# Autodesk Inventor assembly: MultiPass0V_outsideIn-DFMOD
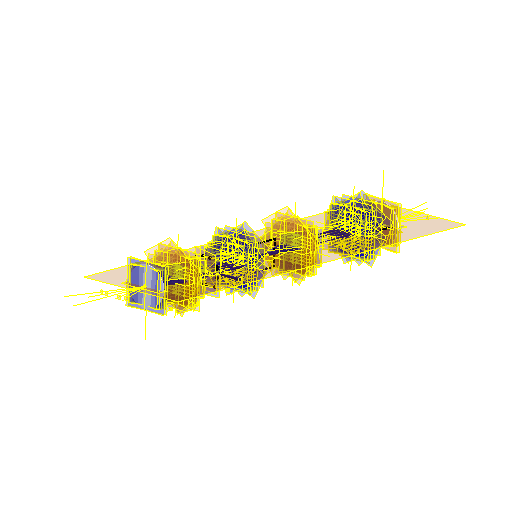
[picture p0: Inventor's stored thumbnail of the model, 512x512]
Saved by Autodesk Inventor 2026.1 (Build 301233000, 233)
## iProperties
Created: 2024-08-19
Part Number: MultiPass0V_outsideIn-DFMOD
Document SubType Name: Assembly
Designer: User
Author: User
## Documents named in this file (14)
- C:\Users\farin012\Downloads\fig4\fig4\MultiPass0V_outsideIn-DFMOD.iam
- C:\Users\farin012\Downloads\fig4\fig4\BB1-E02-Solidworks.ipt
- C:\Users\farin012\Downloads\fig4\fig4\LaserBeamEntry2.ipt
- C:\Users\farin012\Downloads\fig4\fig4\LoopPlane1.ipt
- C:\Users\farin012\Downloads\fig4\fig4\LA1608-AB-Solidworks\LA1608-AB-2LOOP_grid.ipt
- C:\Users\farin012\Downloads\fig4\fig4\LOOP1_COLL.ipt
- C:\Users\farin012\Downloads\fig4\fig4\LOOP1_COLL_L.ipt
- C:\Users\farin012\Downloads\fig4\fig4\LOOP2_COLL.ipt
- C:\Users\farin012\Downloads\fig4\fig4\LOOP2_COLL_L.ipt
- C:\Users\farin012\Downloads\fig4\fig4\LOOP3_COLL.ipt
- C:\Users\farin012\Downloads\fig4\fig4\LOOP3_COLL_L.ipt
- C:\Users\farin012\Downloads\fig4\fig4\deflection_plane.ipt
- C:\Users\farin012\Downloads\fig4\fig4\ExitMirror.ipt
- C:\Users\farin012\Downloads\fig4\fig4\EntryMirror.ipt
## Components (42 placed, 13 different names)
1. BB1-E02-Solidworks:1 — Mate:115, Mate:125, Mate:126, Mate:127, Angle:6, Mate:128, Mate:147, Mate:157, Mate:158, Mate:159, Mate:160
2. BB1-E02-Solidworks:2 — Angle:5, Mate:137, Mate:138, Mate:191
3. LaserBeamEntry2:16 — Mate:124, Flush:7, Mate:179, Mate:180
4. LoopPlane1:1 — Mate:113
5. LA1608-AB-2LOOP_grid:1 — Flush:3, Mate:124, Flush:7, Flush:8, Mate:129, Mate:145, Mate:147, Mate:148, Mate:156, Flush:15, Mate:161, Flush:16
6. LA1608-AB-2LOOP_grid:2 — Flush:2, Flush:9, Mate:130, Mate:136, Mate:145, Mate:146, Mate:149, Mate:155, Flush:14, Mate:162, Flush:17, Mate:164, Mate:174, Flush:22
7. LA1608-AB-2LOOP_grid:3 — Flush:5, Mate:134, Flush:11, Mate:137, Mate:139, Mate:140, Mate:141, Mate:142, Mate:143, Flush:12, Mate:151, Mate:152, Mate:166, Flush:19, Mate:167, Mate:168, Mate:170, Flush:20
8. LA1608-AB-2LOOP_grid:4 — Flush:4, Mate:133, Flush:10, Mate:135, Mate:144, Flush:13, Mate:146, Mate:150, Mate:152, Mate:153, Mate:154, Mate:163, Mate:165, Flush:18, Flush:21
9. LOOP1_COLL:1 — Mate:125, Mate:126
10. LOOP1_COLL:2 — Mate:127, Mate:128
11. LaserBeamEntry2:17 — Flush:8, Mate:129
12. LaserBeamEntry2:18 — Flush:9, Mate:130
13. LOOP1_COLL_L:1 — Mate:135, Mate:136
14. LaserBeamEntry2:19 — Mate:133, Flush:10
15. LaserBeamEntry2:20 — Mate:134, Flush:11
16. LOOP1_COLL:3 — Mate:139, Mate:140
17. LOOP2_COLL:1 — Mate:141, Mate:142
18. LaserBeamEntry2:21 — Mate:144, Flush:13
19. LaserBeamEntry2:22 — Mate:143, Flush:12
20. LOOP2_COLL_L:1 — Mate:153, Mate:154
21. LaserBeamEntry2:23 — Mate:156, Flush:15
22. LaserBeamEntry2:24 — Mate:155, Flush:14
23. LOOP2_COLL:2 — Mate:157, Mate:158
24. LOOP2_COLL:3 — Mate:159, Mate:160
25. LaserBeamEntry2:25 — Mate:161, Flush:16
26. LaserBeamEntry2:26 — Mate:162, Flush:17
27. LOOP2_COLL_L:2 — Mate:163, Mate:164
28. LaserBeamEntry2:27 — Mate:165, Flush:18
29. LaserBeamEntry2:28 — Mate:166, Flush:19
30. LOOP2_COLL:4 — Mate:167, Mate:168
31. LOOP3_COLL:1 — Mate:169, Mate:170
32. LaserBeamEntry2:29 — Mate:172, Flush:21, Mate:188
33. LaserBeamEntry2:30 — Mate:171, Flush:20
34. LOOP3_COLL_L:1 — Mate:173, Mate:174
35. LaserBeamEntry2:31 — Mate:175, Flush:22
36. deflection_plane:1 — Mate:178, Mate:179, Mate:181, Flush:24
37. deflection_plane:2 — Mate:188, Flush:26, Mate:189
38. ExitMirror:1 — Mate:183, Mate:184, Flush:24, Mate:185, Flush:25, Mate:189
39. EntryMirror:1 — Mate:180, Angle:7, Mate:181, Mate:182, Flush:23
40. LaserBeamEntry2:32 — Mate:182, Flush:23
41. LaserBeamEntry2:33 — Mate:185, Flush:25
42. deflection_plane:3 — Mate:190, Angle:8, Mate:191
## Relationships (94: Mate 66, Flush 24, Angle 4)
- Mate:22
- Mate:23
- Mate:113: LoopPlane1:1
- Mate:115: BB1-E02-Solidworks:1
- Angle:5 (180 deg): BB1-E02-Solidworks:2
- Flush:2: LA1608-AB-2LOOP_grid:2
- Flush:3: LA1608-AB-2LOOP_grid:1
- Flush:4: LA1608-AB-2LOOP_grid:4
- Flush:5: LA1608-AB-2LOOP_grid:3
- Mate:124: LaserBeamEntry2:16 ↔ LA1608-AB-2LOOP_grid:1
- Flush:7: LaserBeamEntry2:16 ↔ LA1608-AB-2LOOP_grid:1
- Mate:125: BB1-E02-Solidworks:1 ↔ LOOP1_COLL:1
- Mate:126: BB1-E02-Solidworks:1 ↔ LOOP1_COLL:1
- Mate:127: BB1-E02-Solidworks:1 ↔ LOOP1_COLL:2
- Angle:6 (0 deg): BB1-E02-Solidworks:1
- Mate:128: BB1-E02-Solidworks:1 ↔ LOOP1_COLL:2
- Flush:8: LA1608-AB-2LOOP_grid:1 ↔ LaserBeamEntry2:17
- Mate:129: LA1608-AB-2LOOP_grid:1 ↔ LaserBeamEntry2:17
- Flush:9: LA1608-AB-2LOOP_grid:2 ↔ LaserBeamEntry2:18
- Mate:130: LA1608-AB-2LOOP_grid:2 ↔ LaserBeamEntry2:18
- Mate:133: LA1608-AB-2LOOP_grid:4 ↔ LaserBeamEntry2:19
- Flush:10: LA1608-AB-2LOOP_grid:4 ↔ LaserBeamEntry2:19
- Mate:134: LA1608-AB-2LOOP_grid:3 ↔ LaserBeamEntry2:20
- Flush:11: LA1608-AB-2LOOP_grid:3 ↔ LaserBeamEntry2:20
- Mate:135: LA1608-AB-2LOOP_grid:4 ↔ LOOP1_COLL_L:1
- Mate:136: LA1608-AB-2LOOP_grid:2 ↔ LOOP1_COLL_L:1
- Mate:137 (25 mm): BB1-E02-Solidworks:2 ↔ LA1608-AB-2LOOP_grid:3
- Mate:138: BB1-E02-Solidworks:2
- Mate:139: LA1608-AB-2LOOP_grid:3 ↔ LOOP1_COLL:3
- Mate:140: LA1608-AB-2LOOP_grid:3 ↔ LOOP1_COLL:3
- Mate:141: LA1608-AB-2LOOP_grid:3 ↔ LOOP2_COLL:1
- Mate:142: LA1608-AB-2LOOP_grid:3 ↔ LOOP2_COLL:1
- Mate:143: LA1608-AB-2LOOP_grid:3 ↔ LaserBeamEntry2:22
- Flush:12: LA1608-AB-2LOOP_grid:3 ↔ LaserBeamEntry2:22
- Mate:144: LA1608-AB-2LOOP_grid:4 ↔ LaserBeamEntry2:21
- Flush:13: LA1608-AB-2LOOP_grid:4 ↔ LaserBeamEntry2:21
- Mate:145 (-50 mm): LA1608-AB-2LOOP_grid:1 ↔ LA1608-AB-2LOOP_grid:2
- Mate:146 (50 mm): LA1608-AB-2LOOP_grid:2 ↔ LA1608-AB-2LOOP_grid:4
- Mate:147 (25 mm): BB1-E02-Solidworks:1 ↔ LA1608-AB-2LOOP_grid:1
- Mate:148: LA1608-AB-2LOOP_grid:1
- Mate:149: LA1608-AB-2LOOP_grid:2
- Mate:150: LA1608-AB-2LOOP_grid:4
- Mate:151: LA1608-AB-2LOOP_grid:3
- Mate:152 (-50 mm): LA1608-AB-2LOOP_grid:3 ↔ LA1608-AB-2LOOP_grid:4
- Mate:153: LA1608-AB-2LOOP_grid:4 ↔ LOOP2_COLL_L:1
- Mate:154: LA1608-AB-2LOOP_grid:4 ↔ LOOP2_COLL_L:1
- Mate:155: LA1608-AB-2LOOP_grid:2 ↔ LaserBeamEntry2:24
- Flush:14: LA1608-AB-2LOOP_grid:2 ↔ LaserBeamEntry2:24
- Mate:156: LA1608-AB-2LOOP_grid:1 ↔ LaserBeamEntry2:23
- Flush:15: LA1608-AB-2LOOP_grid:1 ↔ LaserBeamEntry2:23
- Mate:157: BB1-E02-Solidworks:1 ↔ LOOP2_COLL:2
- Mate:158: BB1-E02-Solidworks:1 ↔ LOOP2_COLL:2
- Mate:159: BB1-E02-Solidworks:1 ↔ LOOP2_COLL:3
- Mate:160: BB1-E02-Solidworks:1 ↔ LOOP2_COLL:3
- Mate:161: LA1608-AB-2LOOP_grid:1 ↔ LaserBeamEntry2:25
- Flush:16: LA1608-AB-2LOOP_grid:1 ↔ LaserBeamEntry2:25
- Mate:162: LA1608-AB-2LOOP_grid:2 ↔ LaserBeamEntry2:26
- Flush:17: LA1608-AB-2LOOP_grid:2 ↔ LaserBeamEntry2:26
- Mate:163: LA1608-AB-2LOOP_grid:4 ↔ LOOP2_COLL_L:2
- Mate:164: LA1608-AB-2LOOP_grid:2 ↔ LOOP2_COLL_L:2
- Mate:165: LA1608-AB-2LOOP_grid:4 ↔ LaserBeamEntry2:27
- Flush:18: LA1608-AB-2LOOP_grid:4 ↔ LaserBeamEntry2:27
- Mate:166: LA1608-AB-2LOOP_grid:3 ↔ LaserBeamEntry2:28
- Flush:19: LA1608-AB-2LOOP_grid:3 ↔ LaserBeamEntry2:28
- Mate:167: LA1608-AB-2LOOP_grid:3 ↔ LOOP2_COLL:4
- Mate:168: LA1608-AB-2LOOP_grid:3 ↔ LOOP2_COLL:4
- Mate:169: LOOP3_COLL:1
- Mate:170: LA1608-AB-2LOOP_grid:3 ↔ LOOP3_COLL:1
- Mate:171: LaserBeamEntry2:30
- Flush:20: LA1608-AB-2LOOP_grid:3 ↔ LaserBeamEntry2:30
- Mate:172: LaserBeamEntry2:29
- Flush:21: LA1608-AB-2LOOP_grid:4 ↔ LaserBeamEntry2:29
- Mate:173: LOOP3_COLL_L:1
- Mate:174: LA1608-AB-2LOOP_grid:2 ↔ LOOP3_COLL_L:1
- Mate:175: LaserBeamEntry2:31
- Flush:22: LA1608-AB-2LOOP_grid:2 ↔ LaserBeamEntry2:31
- Mate:178: deflection_plane:1
- Mate:179: LaserBeamEntry2:16 ↔ deflection_plane:1
- Mate:180: LaserBeamEntry2:16 ↔ EntryMirror:1
- Angle:7 (180 deg): EntryMirror:1
- Mate:181: deflection_plane:1 ↔ EntryMirror:1
- Mate:182: EntryMirror:1 ↔ LaserBeamEntry2:32
- Flush:23: EntryMirror:1 ↔ LaserBeamEntry2:32
- Mate:183: ExitMirror:1
- Mate:184: ExitMirror:1
- Flush:24: deflection_plane:1 ↔ ExitMirror:1
- Mate:185: ExitMirror:1 ↔ LaserBeamEntry2:33
- Flush:25: ExitMirror:1 ↔ LaserBeamEntry2:33
- Mate:188 (-25 mm): LaserBeamEntry2:29 ↔ deflection_plane:2
- Flush:26: deflection_plane:2
- Mate:189: deflection_plane:2 ↔ ExitMirror:1
- Mate:190: deflection_plane:3
- Angle:8 (90 deg): deflection_plane:3
- Mate:191 (5 mm): BB1-E02-Solidworks:2 ↔ deflection_plane:3
